# Autodesk Inventor assembly: MecanumFrame2
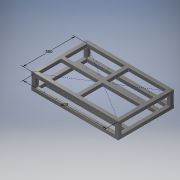
[picture p0: Inventor's stored thumbnail of the model, 180x180]
Saved by Autodesk Inventor 2018 (Build 220112000, 112)
## iProperties
Created: 2017-10-18
Part Number: MecanumFrame2
Document SubType Name: Weldment
Designer: Bryce Richards
Weld Material: Steel, Mild
Mass: 14669.5 g
Surface Area: 23502.9 cm^2
Volume: 1868.72 cm^3
Density: 7.85 g/cm^3
_SolveAssemblyDoc: Frame Generator Solve Assembly
_Version: 15.0.0
Author: Bryce Richards
## Documents named in this file (11)
- C:\Users\P136265\Documents\mecanum-cad\MecanumFrame2.iam
- C:\Users\P136265\Documents\mecanum-cad\MecanumWireframe2.ipt
- C:\Users\P136265\Documents\mecanum-cad\MecanumFrame2\Frame\Frame0001.iam
- C:\Users\P136265\Documents\mecanum-cad\Supports1.ipt
- C:\Users\P136265\Documents\mecanum-cad\Crossmembers.ipt
- C:\Users\P136265\Documents\mecanum-cad\MecanumFrame2\AIP\FEA\caye7aykg.fins
- C:\Users\P136265\Documents\mecanum-cad\MecanumFrame2\AIP\FEA\caye7aykg.fsat
- C:\Users\P136265\Documents\mecanum-cad\MecanumFrame2\AIP\FEA\caye7aykg.ftes
- C:\Users\P136265\Documents\mecanum-cad\MecanumFrame2\AIP\FEA\caye7aykg.fwiz
- C:\Users\P136265\Documents\mecanum-cad\MecanumFrame2\AIP\FEA\caye7ayrk.fmsh
- C:\Users\P136265\Documents\mecanum-cad\MecanumFrame2\AIP\FEA\caye7ayrl.fres
## Components (4 placed, 4 different names)
1. MecanumWireframe2:1
2. Frame0001:1 [sub-assembly]
3. Supports1:1 — Flush:1
4. Crossmembers:1 — Flush:2
## Relationships (2: Flush 2)
- Flush:1: Supports1:1
- Flush:2: Crossmembers:1
## Named parameters: sa_0 = -2.42e-11, sa_1 = 3.87e-11, sa_2 = 588000
note: some values were not read from the file. Shown as the stored number, unit unknown: "sa_0", "sa_1", "sa_2".
